# Autodesk Inventor assembly: Limit switch top + mount left
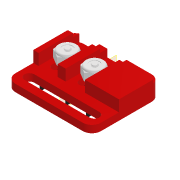
[picture p0: Inventor's stored thumbnail of the model, 180x180]
Saved by Autodesk Inventor 2020 (Build 240168000, 168)
## iProperties
Created: 2019-11-30
Part Number: Limit switch top + mount left
Document SubType Name: Assembly
Designer: ball
Author: ball
## Documents named in this file (5)
- C:\FTC\FTC8863CAD\2019 Robot\Delivery\Lift Right\Limit switch top + mount right.iam
- C:\FTC\FTC8863CAD\Actobotics\605 parts\605630.ipt
- C:\FTC\FTC8863CAD\StepLibraries\Screws\2-56 x .5 TRUSS HEAD PHILLIPS MACHINE SCREW.ipt
- C:\FTC\FTC8863CAD\StepLibraries\Nuts\2-56 NYLON-INSERT LOCKNUT.ipt
- C:\FTC\FTC8863CAD\2019 Robot\Delivery\Lift Right\Limit switch mount top nut well right.ipt
## Components (6 placed, 4 different names)
1. Limit switch mount top nut well right:1 — Mate:8, Angle:1, Mate:10, Angle:2, Mate:12
2. 2-56 x .5 TRUSS HEAD PHILLIPS MACHINE SCREW:1 — Mate:11, Mate:13
3. 2-56 x .5 TRUSS HEAD PHILLIPS MACHINE SCREW:2 — Mate:9, Mate:14
4. 2-56 NYLON-INSERT LOCKNUT:1 — Mate:8, Mate:9, Angle:1
5. 2-56 NYLON-INSERT LOCKNUT:2 — Mate:10, Mate:11, Angle:2
6. 605630:2 — Mate:12, Mate:13, Mate:14
## Relationships (9: Mate 7, Angle 2)
- Mate:8: Limit switch mount top nut well right:1 ↔ 2-56 NYLON-INSERT LOCKNUT:1
- Mate:9: 2-56 x .5 TRUSS HEAD PHILLIPS MACHINE SCREW:2 ↔ 2-56 NYLON-INSERT LOCKNUT:1
- Angle:1 (0 deg): Limit switch mount top nut well right:1 ↔ 2-56 NYLON-INSERT LOCKNUT:1
- Mate:10: Limit switch mount top nut well right:1 ↔ 2-56 NYLON-INSERT LOCKNUT:2
- Mate:11: 2-56 x .5 TRUSS HEAD PHILLIPS MACHINE SCREW:1 ↔ 2-56 NYLON-INSERT LOCKNUT:2
- Angle:2 (0 deg): Limit switch mount top nut well right:1 ↔ 2-56 NYLON-INSERT LOCKNUT:2
- Mate:12: Limit switch mount top nut well right:1 ↔ 605630:2
- Mate:13: 2-56 x .5 TRUSS HEAD PHILLIPS MACHINE SCREW:1 ↔ 605630:2
- Mate:14: 2-56 x .5 TRUSS HEAD PHILLIPS MACHINE SCREW:2 ↔ 605630:2
